# Autodesk Inventor assembly: wheelR802
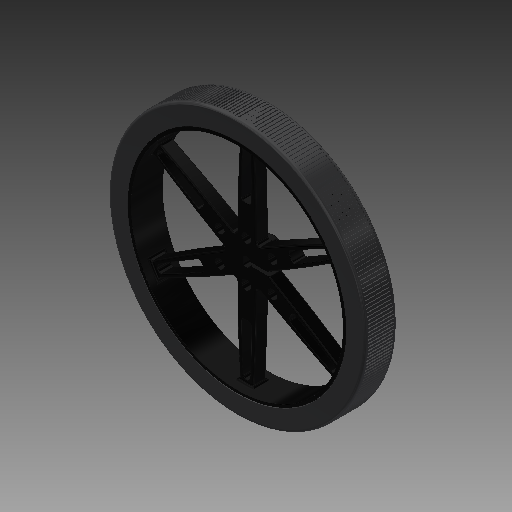
[picture p0: Inventor's stored thumbnail of the model, 512x512]
Saved by Autodesk Inventor 2018 (Build 220112000, 112)
## iProperties
Created: 2019-05-16
Part Number: wheelR802
Material: 一般
Document SubType Name: Assembly
Designer: ku_sk
Mass: 19.7 g
Surface Area: 203.81 cm^2
Volume: 18.5922 cm^3
Author: ku_sk
Sending System: Autodesk Inventor 2018
OS: Windows
FORMAT: text
GUISE: transmit
KEY: wheel
FILE: D:\windows\InventorProjects\Balboa32U4\parts\wheel.x_t
DATE: 2019-May-16 18:05:34
## Documents named in this file (3)
- D:\windows\InventorProjects\Balboa32U4-CAD\parts\wheel\wheelR802.iam
- D:\windows\InventorProjects\Balboa32U4-CAD\parts\wheel\parts\tyre2.ipt
- D:\windows\InventorProjects\Balboa32U4-CAD\parts\wheel\parts\wheel2.ipt
## Components (2 placed, 2 different names)
1. tyre2:1 — 角度:2, メイト:8, メイト:7
2. wheel2:1 — 角度:2, メイト:8, メイト:7, メイト:6, 角度:1, メイト:5
## Relationships (6: Mate 3, Angle 2, Flush 1)
- 角度:2 [Angle] (0 deg): tyre2:1 ↔ wheel2:1
- メイト:8 [Mate]: tyre2:1 ↔ wheel2:1
- メイト:7 [Mate]: tyre2:1 ↔ wheel2:1
- メイト:6 [Flush]: wheel2:1
- 角度:1 [Angle] (-180 deg): wheel2:1
- メイト:5 [Mate]: wheel2:1
